# Autodesk Inventor assembly: Belt Tensioner End_MIR1
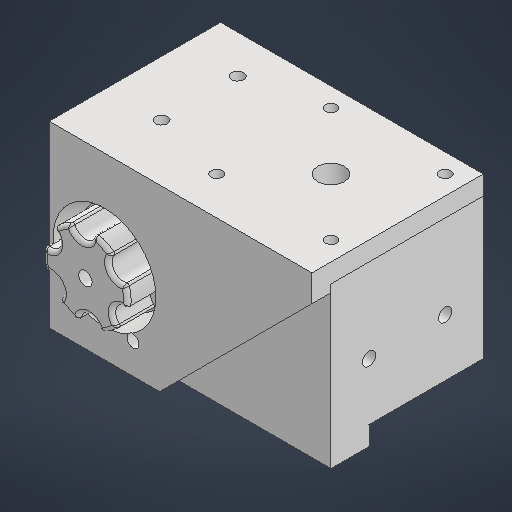
[picture p0: Inventor's stored thumbnail of the model, 512x512]
Saved by Autodesk Inventor 2025.1 (Build 291241000, 241)
## iProperties
Created: 2025-02-02
Part Number: Belt Tensioner End_MIR1
Document SubType Name: Assembly
Designer: jerem
Author: jerem
## Documents named in this file (7)
- C:\Users\jerem\Documents\GitHub\Perovskite-Automated-Synthesis-System\CAD\Gantry\Belt Tensioner End_MIR1.iam
- C:\Users\jerem\Documents\GitHub\Perovskite-Automated-Synthesis-System\CAD\Gantry\Idlert Tensioner_MIR1.ipt
- C:\Users\jerem\Documents\GitHub\Perovskite-Automated-Synthesis-System\CAD\Gantry\tensionerholder_MIR1.ipt
- C:\Users\jerem\Documents\GitHub\Perovskite-Automated-Synthesis-System\CAD\Gantry\X Axis End_MIR2.ipt
- C:\Users\jerem\Documents\GitHub\Perovskite-Automated-Synthesis-System\CAD\Gantry\Tensioner Top_MIR1.ipt
- C:\Users\jerem\Documents\GitHub\Perovskite-Automated-Synthesis-System\CAD\Non 3D Printed Parts\Screws\M3x12_MIR.ipt
- C:\Users\jerem\Documents\GitHub\Perovskite-Automated-Synthesis-System\CAD\Gantry\screw2_MIR.ipt
## Components (6 placed, 6 different names)
1. Idlert Tensioner_MIR1:1 — Angle:1, Mate:8, Angle:2, Mate:10, Mate:9
2. tensionerholder_MIR1:1 — Angle:1, Mate:8, Angle:2, Mate:1, Flush:2, Flush:1, Mate:11
3. X Axis End_MIR2:1 — Mate:1, Flush:2, Flush:1, Mate:7, Mate:6, Mate:5
4. Tensioner Top_MIR1:1 — Mate:7, Mate:6, Mate:5
5. M3x12_MIR:1 — Mate:10, Mate:9, Rotation/Translation:1, Mate:12
6. screw2_MIR:1 — Rotation/Translation:1, Mate:12, Mate:11
## Relationships (14: Mate 9, Angle 2, Flush 2, RelateRotateTranslate 1)
- Angle:1 (180 deg): Idlert Tensioner_MIR1:1 ↔ tensionerholder_MIR1:1
- Mate:8: Idlert Tensioner_MIR1:1 ↔ tensionerholder_MIR1:1
- Angle:2 (0 deg): Idlert Tensioner_MIR1:1 ↔ tensionerholder_MIR1:1
- Mate:1: tensionerholder_MIR1:1 ↔ X Axis End_MIR2:1
- Flush:2: tensionerholder_MIR1:1 ↔ X Axis End_MIR2:1
- Flush:1: tensionerholder_MIR1:1 ↔ X Axis End_MIR2:1
- Mate:7: X Axis End_MIR2:1 ↔ Tensioner Top_MIR1:1
- Mate:6: X Axis End_MIR2:1 ↔ Tensioner Top_MIR1:1
- Mate:5: X Axis End_MIR2:1 ↔ Tensioner Top_MIR1:1
- Mate:10: Idlert Tensioner_MIR1:1 ↔ M3x12_MIR:1
- Mate:9: Idlert Tensioner_MIR1:1 ↔ M3x12_MIR:1
- Rotation/Translation:1 [RelateRotateTranslate] (10.996 mm): M3x12_MIR:1 ↔ screw2_MIR:1
- Mate:12: M3x12_MIR:1 ↔ screw2_MIR:1
- Mate:11: tensionerholder_MIR1:1 ↔ screw2_MIR:1
